# Autodesk Inventor assembly: Z Ring, Sub Assembly
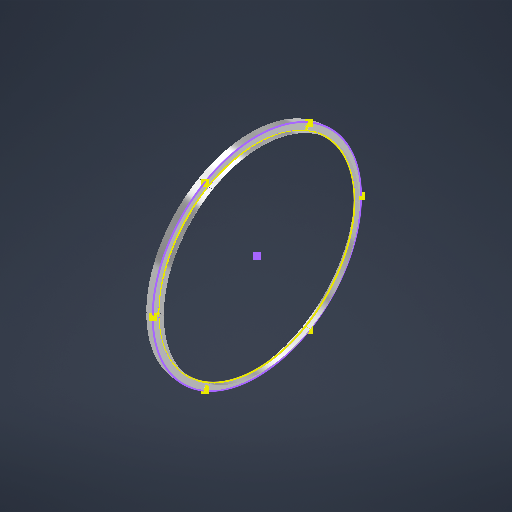
[picture p0: Inventor's stored thumbnail of the model, 512x512]
Saved by Autodesk Inventor 2026.2 (Build 302298000, 298)
## iProperties
Created: 2026-02-02
Part Number: Z Ring, Sub Assembly
Document SubType Name: Assembly
Designer: Lex Machina
Author: Lex Machina
## Documents named in this file (2)
- C:\Users\Lex Machina\GitHub\TSGC-NASA_Senior_Design\CAD\Pressure Vessel\Z Ring, Sub Assembly.iam
- C:\Users\Lex Machina\GitHub\TSGC-NASA_Senior_Design\CAD\Pressure Vessel\Support Ring Section, Z Section.ipt
## Components (6 placed, 1 different names)
1. Support Ring Section, Z Section:1
2. Support Ring Section, Z Section:2
3. Support Ring Section, Z Section:3
4. Support Ring Section, Z Section:4
5. Support Ring Section, Z Section:5
6. Support Ring Section, Z Section:6
## Component patterns: (6 elements, first: Support Ring Section, Z Section:1)
